(part 1 of 2)
# Autodesk Inventor assembly: Rebuild Shooter Assembly
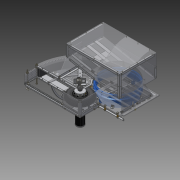
[picture p0: Inventor's stored thumbnail of the model, 180x180]
Saved by Autodesk Inventor 2014 SP1 (Build 180222100, 222)
## iProperties
Created: 2013-10-27
Part Number: Rebuild Shooter Assembly
Document SubType Name: Assembly
Designer: Moses
Mass: 10351.2 g
Surface Area: 36486.6 cm^2
Volume: 5797.69 cm^3
Density: 1.78541 g/cm^3
Author: Moses
## Documents named in this file (107)
- C:\Users\Moses\Documents\Inventor\Rebuilds\Rebuild Sally\Rebuild Shooter Assembly.iam
- C:\Users\Moses\Documents\Inventor\Rebuilds\Rebuild Sally\Spur Gear21.ipt
- C:\Users\Moses\Documents\Inventor\Rebuilds\Rebuild Sally\Bearing Mount 2 v1.ipt
- C:\Users\Moses\Documents\Inventor\Rebuilds\Rebuild Sally\Bearing.ipt
- C:\Users\Moses\Documents\Inventor\Rebuilds\Rebuild Sally\Shorter Shaft.ipt
- C:\Users\Moses\Documents\Inventor\Rebuilds\Rebuild Sally\Rebuild Shooter Main Base.ipt
- C:\Users\Moses\Documents\Inventor\Rebuilds\Rebuild Sally\Gusset 5.ipt
- C:\Users\Moses\Documents\Inventor\Rebuilds\Rebuild Sally\Rebuild L-Channel Strength.ipt
- C:\Users\Moses\Documents\Inventor\Rebuilds\Rebuild Sally\Bearing Mount v1.ipt
- C:\Users\Moses\Documents\Inventor\Rebuilds\Rebuild Sally\Bearing Mount Top.ipt
- C:\Users\Moses\Documents\Inventor\Rebuilds\Rebuild Sally\Rubber Cushion.ipt
- C:\Users\Moses\Documents\Inventor\Rebuilds\Rebuild Sally\CIM Bearing.ipt
- C:\Users\Moses\Documents\Inventor\Rebuilds\Rebuild Sally\Pneumatic Wheel.iam
- C:\Users\Moses\Documents\Inventor\Rebuilds\Rebuild Sally\2469K200.ipt
- C:\Users\Moses\Documents\Inventor\Rebuilds\Rebuild Sally\CIM motor1.ipt
- C:\Users\Moses\Documents\Inventor\Rebuilds\Rebuild Sally\Cim Mount.ipt
- C:\Users\Moses\Documents\Inventor\Rebuilds\Rebuild Sally\Runner Rails v2.ipt
- C:\Users\Moses\Documents\Inventor\Rebuilds\Rebuild Sally\Pneumatic Hub.ipt
- C:\Users\Moses\Documents\Inventor\Rebuilds\Rebuild Sally\0.25x20 Washer.ipt
- C:\Users\Moses\Documents\Inventor\Rebuilds\Rebuild Sally\Standard High-Strength Steel Cap Screw 0.25-20 Thread\Fully Threaded\1.000 in 92620A542\92620A542.ipt
- C:\Users\Moses\Documents\Inventor\Rebuilds\Rebuild Sally\Standard High-Strength Steel Cap Screw 0.25-20 Thread\90630A110.ipt
- C:\Users\Moses\Documents\Inventor\Rebuilds\Rebuild Sally\Standard High-Strength Steel Cap Screw 0.25-20 Thread\Fully Threaded\6.000 in 92620A559\92620A559.ipt
- C:\Users\Moses\Documents\Inventor\Rebuilds\Rebuild Sally\8mm shaft 2.ipt
- C:\Users\Moses\Documents\Inventor\Rebuilds\Rebuild Sally\93330A493.ipt
- C:\Users\Moses\Documents\Inventor\Rebuilds\Rebuild Sally\Standard High-Strength Steel Cap Screw 0.25-20 Thread\Fully Threaded\5.000 in 92620A557\92620A557.ipt
- C:\Users\Moses\Documents\Inventor\Rebuilds\Rebuild Sally\6280K341.ipt
- C:\Users\Moses\Documents\Inventor\Rebuilds\Rebuild Sally\0.5 inch Shaft to 8mm Shaft Insert.ipt
- C:\Users\Moses\Documents\Inventor\Rebuilds\Rebuild Sally\8mm Shaft Spacer 1 Shooter.ipt
- C:\Users\Moses\Documents\Inventor\Rebuilds\Rebuild Sally\Shooter 8mm Key Sprocket Encoder.ipt
- C:\Users\Moses\Documents\Inventor\Rebuilds\Rebuild Sally\Standard High-Strength Steel Cap Screw 0.25-20 Thread\Fully Threaded\4.000 in 92620A555\92620A555.ipt
- C:\Users\Moses\Documents\Inventor\Rebuilds\Rebuild Sally\Shooter Side Support Bar - R.ipt
- C:\Users\Moses\Documents\Inventor\Rebuilds\Rebuild Sally\Shooter Side Support Bar - L.ipt
- C:\Users\Moses\Documents\Inventor\Rebuilds\Rebuild Sally\Shooter Back Support Bar.ipt
- C:\Users\Moses\Documents\Inventor\Rebuilds\Rebuild Sally\Shooter Middle Support Bar.ipt
- C:\Users\Moses\Documents\Inventor\Rebuilds\Rebuild Sally\Drive Base Kit\DBK_0820Spacer_am-2243 (modified).ipt
- C:\Users\Moses\Documents\Inventor\Rebuilds\Rebuild Sally\Drive Base Kit\DBK_0820Spacer_am-2243 (modified 2).ipt
- C:\Users\Moses\Documents\Inventor\Rebuilds\Rebuild Sally\Standard #10 Washer.ipt
- C:\Users\Moses\Documents\Inventor\Rebuilds\Rebuild Sally\10-32 316 Stainless Steel Pan Head Philips Machine Screw\0.500\91735A829.ipt
- C:\Users\Moses\Documents\Inventor\Rebuilds\Rebuild Sally\Wheel Shield 1.ipt
- C:\Users\Moses\Documents\Inventor\Rebuilds\Rebuild Sally\Wheel Shield 2.ipt
- C:\Users\Moses\Documents\Inventor\Rebuilds\Rebuild Sally\Standard High-Strength Steel Cap Screw 0.25-20 Thread\Fully Threaded\1.500 in 92620A546\92620A546.ipt
- C:\Users\Moses\Documents\Inventor\Rebuilds\Rebuild Sally\Standard High-Strength Steel Cap Screw 0.25-20 Thread\Fully Threaded\1.250 in 92620A544\92620A544.ipt
- C:\Users\Moses\Documents\Inventor\Rebuilds\Rebuild Sally\Standard High-Strength Steel Cap Screw 0.25-20 Thread\Fully Threaded\1.750 in 92620A548\92620A548.ipt
- C:\Users\Moses\Documents\Inventor\Rebuilds\Rebuild Sally\0.25x20 Washer Large Diameter.ipt
- C:\Users\Moses\Documents\Inventor\Rebuilds\Rebuild Sally\7547K130.ipt
- C:\Users\Moses\Documents\Inventor\Rebuilds\Rebuild Sally\Hopper Bracing P1.ipt
- C:\Users\Moses\Documents\Inventor\Rebuilds\Rebuild Sally\Shooter I Brace.ipt
- C:\Users\Moses\Documents\Inventor\Rebuilds\Rebuild Sally\Standard High-Strength Steel Cap Screw 0.25-20 Thread\Fully Threaded\0.750 in 92620A540\92620A540.ipt
- C:\Users\Moses\Documents\Inventor\Rebuilds\Rebuild Sally\Standard High-Strength Steel Cap Screw 0.25-20 Thread\Thread Length 0.75 - 1 in\1.250 in 91257A544\91257A544.ipt
- C:\Users\Moses\Documents\Inventor\Rebuilds\Rebuild Sally\Rebuild Outer Rail v1.ipt
- C:\Users\Moses\Documents\Inventor\Rebuilds\Rebuild Sally\Standard High-Strength Steel Cap Screw 0.25-20 Thread\Fully Threaded\0.500 in 92620A537\92620A537.ipt
- C:\Users\Moses\Documents\Inventor\Rebuilds\Rebuild Sally\91831A411.ipt
- C:\Users\Moses\Documents\Inventor\Rebuilds\Rebuild Sally\10-32 316 Stainless Steel Pan Head Philips Machine Screw\0.750\91735A831.ipt
- C:\Users\Moses\Documents\Inventor\Rebuilds\Rebuild Sally\Shooter Magnetic Sensor Mount Bracket.ipt
- C:\Users\Moses\Documents\Inventor\Rebuilds\Rebuild Sally\176_DP_D_229__F_D_231_1__F_D_3556__2_03\7.ipt
- C:\Users\Moses\Documents\Inventor\Rebuilds\Rebuild Sally\Shooter Top Shield.ipt
- C:\Users\Moses\Documents\Inventor\Rebuilds\Rebuild Sally\Shooter Wheel Shields Connector Bar.ipt
- C:\Users\Moses\Documents\Inventor\Rebuilds\Rebuild Sally\Drive Base Kit\DBK_0820Spacer_am-2243 (modified 3).ipt
- C:\Users\Moses\Documents\Inventor\Rebuilds\Rebuild Sally\0.125 Pop Rivet.ipt
- C:\Users\Moses\Documents\Inventor\Rebuilds\Rebuild Sally\Shooter Magnetic Sensor V2.ipt
- C:\Users\Moses\Documents\Inventor\Rebuilds\Rebuild Sally\Hopper Bracing P2.ipt
- C:\Users\Moses\Documents\Inventor\Rebuilds\Rebuild Sally\Hopper Bracing P3.ipt
- C:\Users\Moses\Documents\Inventor\Rebuilds\Rebuild Sally\Hopper Left Side Leg.ipt
- C:\Users\Moses\Documents\Inventor\Rebuilds\Rebuild Sally\Hopper Right Side Leg.ipt
- C:\Users\Moses\Documents\Inventor\Rebuilds\Rebuild Sally\Hopper Bottom.ipt
- C:\Users\Moses\Documents\Inventor\Rebuilds\Rebuild Sally\Hopper Left Side.ipt
- C:\Users\Moses\Documents\Inventor\Rebuilds\Rebuild Sally\Hopper Back Wedge Side.ipt
- C:\Users\Moses\Documents\Inventor\Rebuilds\Rebuild Sally\Hopper Top.ipt
- C:\Users\Moses\Documents\Inventor\Rebuilds\Rebuild Sally\Hopper Bracing Top Left P4.ipt
- C:\Users\Moses\Documents\Inventor\Rebuilds\Rebuild Sally\Hopper Front.ipt
- C:\Users\Moses\Documents\Inventor\Rebuilds\Rebuild Sally\Hopper Right.ipt
- C:\Users\Moses\Documents\Inventor\Rebuilds\Rebuild Sally\Hopper Bracing Front Left P5.ipt
- C:\Users\Moses\Documents\Inventor\Rebuilds\Rebuild Sally\Hopper Bracing Front Bottom P6.ipt
- C:\Users\Moses\Documents\Inventor\Rebuilds\Rebuild Sally\Hopper Bracing Front Right P7.ipt
- C:\Users\Moses\Documents\Inventor\Rebuilds\Rebuild Sally\Hopper Bracing Front Top P8.ipt
- C:\Users\Moses\Documents\Inventor\Rebuilds\Rebuild Sally\Hopper Bracing Right Bottom P9.ipt
- C:\Users\Moses\Documents\Inventor\Rebuilds\Rebuild Sally\Hopper Bracing Right Top P10.ipt
- C:\Users\Moses\Documents\Inventor\Rebuilds\Rebuild Sally\Hopper Teflon Strip P1.ipt
- C:\Users\Moses\Documents\Inventor\Rebuilds\Rebuild Sally\Hopper Teflon Strip P2.ipt
- C:\Users\Moses\Documents\Inventor\Rebuilds\Rebuild Sally\Hopper Teflon Strip P3.ipt
- C:\Users\Moses\Documents\Inventor\Rebuilds\Rebuild Sally\Hopper Teflon Strip P4.ipt
- C:\Users\Moses\Documents\Inventor\Rebuilds\Rebuild Sally\Hopper Bracing Back Bottom P11.ipt
- C:\Users\Moses\Documents\Inventor\Rebuilds\Rebuild Sally\Hopper Bracing Back Left P12.ipt
- C:\Users\Moses\Documents\Inventor\Rebuilds\Rebuild Sally\Hopper Bracing Right Leg P13.ipt
- C:\Users\Moses\Documents\Inventor\Rebuilds\Rebuild Sally\Hopper Bouncer Mounting Brace P1.ipt
- C:\Users\Moses\Documents\Inventor\Rebuilds\Rebuild Sally\Bounce Polycarbonate Flap.ipt
- C:\Users\Moses\Documents\Inventor\Rebuilds\Rebuild Sally\Hopper Bracing P12 to P1.ipt
- C:\Users\Moses\Documents\Inventor\Rebuilds\Rebuild Sally\Hopper Pail Mounting Brace P13.ipt
- C:\Users\Moses\Documents\Inventor\Rebuilds\Rebuild Sally\Trimmed Leaktite 3.5-Gal. Blue Plastic Translucent Pail Hopper V3.ipt
- C:\Users\Moses\Documents\Inventor\Rebuilds\Rebuild Sally\Hopper Teflon Strip P5.ipt
- C:\Users\Moses\Documents\Inventor\Rebuilds\Rebuild Sally\Hopper Teflon Strip P6.ipt
- C:\Users\Moses\Documents\Inventor\Rebuilds\Rebuild Sally\Hopper to Pail Polycarbonate Flap Connector V2.ipt
- C:\Users\Moses\Documents\Inventor\Rebuilds\Rebuild Sally\90715A007.ipt
- C:\Users\Moses\Documents\Inventor\Rebuilds\Rebuild Sally\Drive Base Kit\DBK_0820Spacer_am-2243 (modified for Shooter Shaft Spacer 1).ipt
- C:\Users\Moses\Documents\Inventor\Rebuilds\Rebuild Sally\Drive Base Kit\DBK_0820Spacer_am-2243 (modified for Shooter Shaft Spacer 2).ipt
- C:\Users\Moses\Documents\Inventor\Rebuilds\Rebuild Sally\10-32 Black-Oxide Alloy Steel Socket Head Cap Screw\0.7500\91251A345.ipt
- C:\Users\Moses\Documents\Inventor\Rebuilds\Rebuild Sally\10-32 Black-Oxide Alloy Steel Socket Head Cap Screw\2.5000\91251A355.ipt
- C:\Users\Moses\Documents\Inventor\Rebuilds\Rebuild Sally\Shooter 8mm Key Primary Wheel.ipt
- C:\Users\Moses\Documents\Inventor\Rebuilds\Rebuild Sally\Rebuild Shooter NCDME075-0600 Cylinder Mounting Bracket.ipt
- C:\Users\Moses\Documents\Inventor\Rebuilds\Rebuild Sally\NCDME075-0600 SMC Pneumatic Cylinder.iam
- C:\Users\Moses\Documents\Inventor\Rebuilds\Rebuild Sally\94846A535.ipt
- C:\Users\Moses\Documents\Inventor\Rebuilds\Rebuild Sally\Rebuild Puller Hook.ipt
- C:\Users\Moses\Documents\Inventor\Rebuilds\Rebuild Sally\Standard #4 Washer.ipt
- C:\Users\Moses\Documents\Inventor\Rebuilds\Rebuild Sally\4-40 18-8 Stainless Steel Pan Head Phillips Machine Screw\18-8 Stainless Steel Nylon-Insert Hex Locknut\91831A005.ipt
- C:\Users\Moses\Documents\Inventor\Rebuilds\Rebuild Sally\4-40 18-8 Stainless Steel Pan Head Phillips Machine Screw\0.6250\91772A112.ipt
- C:\Users\Moses\Documents\Inventor\Rebuilds\Rebuild Sally\4-40 18-8 Stainless Steel Pan Head Phillips Machine Screw\0.5000\91772A110.ipt
- C:\Users\Moses\Documents\Inventor\Rebuilds\Rebuild Sally\4-40 18-8 Stainless Steel Pan Head Phillips Machine Screw\0.7500\91772A113.ipt
## Components (473 placed, 106 different names)
1. Shooter Wheel Shields Connector Bar:1 — Mate:124, Mate:125, Flush:76, Mate:89, Mate:128
2. Shooter Top Shield:1 — Flush:73, Mate:123, Flush:74, Flush:75, Insert:58, Insert:57, Mate:119, Mate:188, Flush:163
3. Shooter Magnetic Sensor Mount Bracket:1 — Mate:119, Angle:74, Mate:120, Mate:121, Insert:177, Insert:178
4. DBK_0820Spacer_am-2243 (modified 3):1 — Insert:196
5. 93330A493:1 — Insert:75
6. 7547K130:3 — Mate:101, Mate:102, Mate:103
7. 7547K130:1 — Mate:98, Mate:99, Mate:100
8. Shooter I Brace:1 — Mate:105, Flush:18, Mate:109, Mate:111, Mate:113, Flush:175, Insert:390, Insert:392, Insert:393, Insert:394
9. Shooter Side Support Bar - R:1 — Mate:84, Tangent:86, Flush:6, Mate:86, Flush:8, Insert:78, Insert:114, Insert:115, Insert:135
10. Shooter Side Support Bar - L:1 — Mate:85, Flush:7, Tangent:87, Insert:92, Insert:100, Mate:128, Insert:305, Insert:361, Mate:228, Mate:229, Flush:176
11. Shooter Middle Support Bar:1 — Flush:14, Mate:93, Insert:85, Insert:87, Mate:57, Insert:45, Insert:103, Insert:104, Insert:164
12. Shooter Back Support Bar:1 — Mate:86, Tangent:88, Flush:8, Mate:40, Insert:130, Flush:151, Flush:174
13. Wheel Shield 2:1 — Mate:89, Flush:10, Mate:90, Flush:11, Mate:124, Flush:76, Insert:201, Insert:202
14. Wheel Shield 1:1 — Mate:88, Flush:9, Flush:10, Mate:90, Flush:11, Mate:125, Insert:199, Insert:200
15. Rubber Cushion:1 — Mate:48, Mate:49, Flush:3
16. Bearing:2 — Mate:19, Mate:103
17. Bearing:1 — Mate:100
18. Spur Gear2:1 — Mate:20, Mate:21, Mate:22, Mate:23, Mate:24, Mate:25, Mate:27, Mate:28, Mate:29, Mate:30, Mate:31, Mate:32, Insert:395, Insert:396
19. Shorter Shaft:1 — Mate:19, Mate:98, Mate:99, Mate:101, Mate:102
20. Runner Rails v2:1 — Mate:59, Mate:60, Mate:61, Insert:84, Flush:14, Insert:86, Insert:88, Insert:101, Insert:102, Mate:104, Mate:220, Flush:17, Insert:171, Insert:172, Insert:173, Insert:174, Insert:175, Insert:176, Mate:130, Mate:132, Flush:78, Mate:133, Mate:135, Mate:152, Mate:200, Tangent:94, Flush:165, Mate:202, Mate:205, Mate:206, Mate:221
21. Cim Mount:1 — Insert:9, Mate:55, Mate:56, Mate:57, Mate:58, Insert:22, Insert:23, Insert:34, Insert:35, Insert:40, Insert:71, Insert:72, Insert:75, Mate:93, Insert:93, Insert:116, Insert:117, Insert:163, Insert:363, Insert:364
22. Bearing Mount Top:1 — Mate:45, Mate:46, Mate:47, Insert:7, Mate:50, Insert:56, Angle:74, Mate:120, Mate:121, Mate:122, Flush:73, Mate:123, Flush:74, Flush:75, Mate:153
23. Rebuild Outer Rail v1:1 — Mate:42, Mate:44, Mate:45, Mate:46, Mate:48, Insert:51, Insert:53, Insert:55, Insert:69, Mate:114, Flush:65, Flush:66
24. Rebuild Outer Rail v1:2 — Mate:114, Flush:65, Flush:66, Mate:115, Flush:67, Flush:70
25. Rebuild Outer Rail v1:3 — Mate:115, Mate:116, Flush:67, Flush:68, Flush:70, Flush:71
26. Rebuild Outer Rail v1:4 — Mate:116, Mate:117, Flush:68, Flush:69, Flush:71, Flush:72
27. Rebuild Outer Rail v1:5 — Mate:117, Flush:69, Flush:72, Mate:118, Mate:222
28. Bearing Mount v1:1 — Mate:39, Mate:40, Flush:2, Mate:41, Mate:44, Mate:49, Flush:3, Insert:8, Mate:59, Mate:60, Mate:61, Insert:66, Insert:94, Mate:118, Insert:165, Insert:166, Insert:167, Insert:168, Insert:169, Insert:170
29. Rebuild L-Channel Strength:1 — Mate:36, Mate:37, Mate:38, Mate:88, Flush:9, Insert:121, Insert:125, Mate:127, Insert:208, Insert:303, Insert:304
30. Gusset 5:4 — Mate:27, Mate:31, Mate:32, Insert:146, Insert:153
31. Gusset 5:3 — Mate:28, Mate:29, Mate:30, Mate:33, Insert:141, Insert:152
32. Gusset 5:2 — Mate:23, Mate:24, Mate:25, Mate:34, Mate:35, Insert:145, Insert:150
33. Gusset 5:1 — Mate:20, Mate:21, Mate:22, Insert:147, Insert:151
34. Bearing Mount 2 v1:1 — Mate:8, Mate:9, Mate:10, Mate:14, Insert:139
35. Bearing Mount 2 v1:2 — Mate:11, Mate:12, Mate:13, Insert:133, Insert:137
36. Rebuild Shooter Main Base:1 — Mate:11, Mate:12, Mate:8, Mate:9, Mate:10, Mate:13, Mate:14, Mate:33, Mate:34, Mate:35, Mate:36, Mate:37, Mate:38, Mate:39, Flush:2, Mate:41, Mate:42, Mate:55, Mate:56, Insert:65, Mate:74, Insert:76, Mate:84, Flush:6, Mate:85, Flush:7, Insert:44, Insert:112, Insert:122, Mate:105, Flush:18, Insert:148, Insert:149, Mate:106, Mate:107, Mate:108, Mate:110, Mate:112, Mate:126, Insert:196, Insert:207, Insert:39, Angle:79, Angle:80
37. Shooter 8mm Key Primary Wheel:1 — Flush:173, Mate:225, Mate:226, Mate:227
38. DBK_0820Spacer_am-2243 (modified for Shooter Shaft Spacer 1):1 — Insert:358
39. DBK_0820Spacer_am-2243 (modified for Shooter Shaft Spacer 2):1 — Insert:359
40. Shooter Magnetic Sensor V2:1 — Insert:177
41. 6280K341:1 — Mate:77, Flush:5, Angle:3, Mate:78
42. 0.5 inch Shaft to 8mm Shaft Insert:1 — Mate:75, Mate:76, Mate:77, Flush:5, Angle:3
43. 8mm Shaft Spacer 1 Shooter:1 — Mate:79, Mate:80, Mate:78, Mate:83
44. Shooter 8mm Key Sprocket Encoder:1 — Mate:81, Mate:82, Mate:83
45. 8mm shaft 2:1 — Mate:51, Mate:52, Mate:54, Rotation:1, Mate:66, Mate:67, Mate:68, Mate:69, Mate:75, Mate:76, Mate:79, Mate:81, Mate:82, Mate:226
46. Pneumatic Wheel:1 [sub-assembly] — Mate:50, Mate:70, Mate:71, Mate:72
47. 2469K200:1 — Mate:52, Mate:53, Flush:4, Rotation:1
48. CIM motor1:1 — Mate:53, Mate:54, Flush:4, Insert:9, Mate:58
49. Pneumatic Hub:1 — Mate:66, Mate:69, Mate:71, Insert:368, Insert:374, Insert:375, Insert:376, Insert:377, Insert:378
50. Pneumatic Hub:2 — Mate:67, Mate:68, Mate:70, Mate:72, Insert:188, Insert:189, Insert:190, Insert:191, Insert:192, Insert:193, Mate:122, Insert:359, Flush:173, Mate:225, Mate:227
51. CIM Bearing:2 — Insert:8, Insert:358
52. CIM Bearing:1 — Insert:7, Mate:51, Mate:80
53. 90630A110:37 — Insert:391
54. 0.25x20 Washer:100 — Insert:127, Insert:392
55. 0.25x20 Washer:102 — Insert:129, Insert:394
56. 0.25x20 Washer:101 — Insert:128, Insert:393
57. Standard #4 Washer:1 — Insert:395, Insert:398
58. Standard #4 Washer:2 — Insert:396, Insert:397
59. 91772A112:1 — Insert:398
60. 91831A005:1 — Insert:397
61. 90630A110:36
62. 0.25x20 Washer:98 — Insert:388
63. 91257A544:5 — Insert:389
64. 0.25x20 Washer:99 — Insert:389, Insert:390
65. 94846A535:1 — Insert:386
66. 91831A005:8 — Insert:379
67. Standard #4 Washer:14 — Insert:379
68. 91831A005:7 — Insert:380
69. Standard #4 Washer:13 — Insert:380
70. 91772A113:2
71. 91772A113:1
72. Standard #10 Washer:12 — Insert:364, Insert:365
73. Standard #10 Washer:13 — Insert:363, Insert:366
74. 91251A345:1 — Insert:366
75. 91251A345:2 — Insert:365
76. 91251A355:1 — Insert:367
77. Standard #10 Washer:14 — Insert:367, Insert:368
78. 91251A355:2
79. Standard #10 Washer:15 — Insert:374
80. 91251A355:3
81. Standard #10 Washer:16 — Insert:375
82. 91251A355:4
83. Standard #10 Washer:17 — Insert:376
84. 91251A355:5
85. 91251A355:6
86. Standard #10 Washer:18 — Insert:378
87. Standard #10 Washer:19 — Insert:377
88. DBK_0820Spacer_am-2243 (modified):1 — Insert:89, Mate:92
89. DBK_0820Spacer_am-2243 (modified 2):1 — Insert:91
90. DBK_0820Spacer_am-2243 (modified):2 — Insert:90
91. DBK_0820Spacer_am-2243 (modified 2):2 — Insert:362
92. 91257A544:4
93. 0.25x20 Washer:97 — Insert:361
94. 0.125 Pop Rivet:91 — Mate:224, Tangent:211
95. 91831A005:13 — Insert:303
96. 91831A005:14 — Insert:304
97. 91772A110:8
98. 90715A007:3 — Insert:305
99. 91772A110:9
100. 91772A110:10
101. 91831A005:15 — Insert:309
102. Standard #4 Washer:33 — Insert:309
103. 91831A005:16 — Insert:310
104. Standard #4 Washer:34 — Insert:310
105. 91831A005:17 — Insert:313
106. Standard #4 Washer:35 — Insert:313
107. 91831A005:18 — Insert:314
108. Standard #4 Washer:36 — Insert:314
109. 91831A005:19 — Insert:315
110. Standard #4 Washer:37 — Insert:315
111. 91772A112:4
112. 91772A112:5
113. 91772A112:6
114. 91772A112:7
115. 91772A112:8
116. 91831A005:9 — Insert:324
117. Standard #4 Washer:20 — Insert:324, Insert:328
118. 91831A005:10 — Insert:325
119. Standard #4 Washer:21 — Insert:325, Insert:329
120. 91831A005:11 — Insert:326
121. Standard #4 Washer:22 — Insert:326, Insert:330
122. 91831A005:12 — Insert:327
123. Standard #4 Washer:23 — Insert:327, Insert:331
124. 91772A110:7
125. 91772A110:6
126. 91772A110:5
127. 91772A110:4
128. 91257A544:3 — Insert:336
129. 91831A005:4 — Insert:337
130. Standard #4 Washer:5 — Insert:337, Insert:340
131. 91831A005:5 — Insert:338
132. Standard #4 Washer:4 — Insert:338, Insert:341
133. 91831A005:6 — Insert:339
134. Standard #4 Washer:3 — Insert:339, Insert:342
135. 91772A110:1
136. 91772A110:2
137. 91772A110:3
138. 91831A005:2 — Insert:346
139. Standard #4 Washer:11 — Insert:346
140. 91831A005:3 — Insert:348
141. Standard #4 Washer:12 — Insert:348
142. 91772A112:2
143. 91831A005:21
144. 91772A112:3
145. Standard #4 Washer:39
146. 91831A005:20
147. Standard #4 Washer:38
148. 91772A112:10
149. 91772A112:9
150. 0.125 Pop Rivet:90 — Mate:217, Tangent:209
151. 0.125 Pop Rivet:87 — Insert:302, Mate:218
152. 0.125 Pop Rivet:88 — Insert:301, Mate:219
153. 0.125 Pop Rivet:89 — Mate:216, Tangent:208
154. 0.125 Pop Rivet:85 — Insert:299, Mate:205
155. 0.125 Pop Rivet:86 — Insert:300
156. 0.125 Pop Rivet:78 — Insert:292, Mate:197
157. 0.125 Pop Rivet:79 — Insert:293
158. 0.125 Pop Rivet:81 — Insert:295
159. 0.125 Pop Rivet:80 — Insert:294, Mate:198
160. 0.125 Pop Rivet:82 — Insert:296
161. 0.125 Pop Rivet:84 — Insert:297
162. 0.125 Pop Rivet:83 — Insert:298
163. Standard #4 Washer:6 — Insert:277
164. Standard #4 Washer:7 — Insert:278
165. Standard #4 Washer:8 — Insert:279
166. Standard #4 Washer:10
167. Standard #4 Washer:9
168. Standard #4 Washer:30
169. Standard #4 Washer:32
170. Standard #4 Washer:31 — Insert:284
171. Standard #4 Washer:29 — Insert:286
172. Standard #4 Washer:25
173. Standard #4 Washer:26
174. Standard #4 Washer:27
175. Standard #4 Washer:28 — Insert:291
176. Standard #4 Washer:24 — Insert:290
177. 0.125 Pop Rivet:76 — Insert:275
178. 0.125 Pop Rivet:77 — Insert:276
179. 0.125 Pop Rivet:68 — Insert:267
180. 0.125 Pop Rivet:69 — Insert:268
181. 0.125 Pop Rivet:70 — Insert:269
182. 0.125 Pop Rivet:71 — Insert:270
183. 0.125 Pop Rivet:72 — Insert:271
184. 0.125 Pop Rivet:73 — Insert:272
185. 0.125 Pop Rivet:75 — Insert:274
186. 0.125 Pop Rivet:74 — Insert:273
187. 0.125 Pop Rivet:47 — Mate:179, Tangent:92
188. 0.125 Pop Rivet:46 — Mate:178, Tangent:93
189. 0.125 Pop Rivet:48 — Mate:180, Tangent:91
190. 0.125 Pop Rivet:49 — Mate:181, Tangent:90
191. 0.125 Pop Rivet:50 — Mate:182, Tangent:89
192. 0.125 Pop Rivet:52 — Insert:251
193. 0.125 Pop Rivet:51 — Insert:250
194. 0.125 Pop Rivet:53 — Insert:252
195. 0.125 Pop Rivet:54 — Insert:253
196. 0.125 Pop Rivet:55 — Insert:254
197. 0.125 Pop Rivet:57 — Insert:256
198. 0.125 Pop Rivet:56 — Insert:255
199. 0.125 Pop Rivet:59 — Insert:258
200. 0.125 Pop Rivet:58 — Insert:257
201. 0.125 Pop Rivet:61 — Insert:260
202. 0.125 Pop Rivet:60 — Insert:259
203. 0.125 Pop Rivet:63 — Insert:262
204. 0.125 Pop Rivet:62 — Insert:261
205. 0.125 Pop Rivet:64 — Insert:263
206. 0.125 Pop Rivet:65 — Insert:264
207. 0.125 Pop Rivet:67 — Insert:266
208. 0.125 Pop Rivet:66 — Insert:265
209. 0.125 Pop Rivet:23 — Insert:227
210. 0.125 Pop Rivet:24 — Insert:228
211. 0.125 Pop Rivet:25 — Insert:229
212. 0.125 Pop Rivet:26 — Insert:230
213. 0.125 Pop Rivet:27 — Insert:231
214. 0.125 Pop Rivet:29 — Insert:233
215. 0.125 Pop Rivet:28 — Insert:232
216. 0.125 Pop Rivet:30 — Insert:234
217. 0.125 Pop Rivet:31 — Insert:235
218. 0.125 Pop Rivet:32 — Insert:236
219. 0.125 Pop Rivet:34 — Insert:238
220. 0.125 Pop Rivet:33 — Insert:237
221. 0.125 Pop Rivet:35 — Insert:239
222. 0.125 Pop Rivet:36 — Insert:240
223. 0.125 Pop Rivet:37 — Insert:241
224. 0.125 Pop Rivet:38 — Insert:242
225. 0.125 Pop Rivet:39 — Insert:243
226. 0.125 Pop Rivet:40 — Insert:244
227. 0.125 Pop Rivet:41 — Insert:245
228. 0.125 Pop Rivet:42 — Insert:246
229. 0.125 Pop Rivet:43 — Insert:247
230. 0.125 Pop Rivet:44 — Insert:248
231. 0.125 Pop Rivet:45 — Insert:249
232. 0.125 Pop Rivet:19 — Insert:223
233. 0.125 Pop Rivet:20 — Insert:224
234. 0.125 Pop Rivet:21 — Insert:225
235. 0.125 Pop Rivet:22 — Insert:226
236. 0.125 Pop Rivet:11 — Insert:215
237. 0.125 Pop Rivet:12 — Insert:216
238. 0.125 Pop Rivet:13 — Insert:217
239. 0.125 Pop Rivet:15 — Insert:219
240. 0.125 Pop Rivet:14 — Insert:218
241. 0.125 Pop Rivet:16 — Insert:220
242. 0.125 Pop Rivet:17 — Insert:221
243. 0.125 Pop Rivet:18 — Insert:222
244. 0.125 Pop Rivet:6 — Insert:210
245. 0.125 Pop Rivet:7 — Insert:211
246. 0.125 Pop Rivet:8 — Insert:212
247. 0.125 Pop Rivet:9 — Insert:213
248. 0.125 Pop Rivet:10 — Insert:214
249. 90630A110:35 — Insert:208
250. 0.25x20 Washer:96 — Insert:207, Insert:209
251. 92620A540:11 — Insert:209
252. Standard #4 Washer:40
253. Standard #4 Washer:41
254. 0.25x20 Washer:95 — Mate:126, Mate:127, Insert:194
255. 90630A110:34 — Insert:194
256. 92620A540:10 — Insert:195
257. Standard #4 Washer:18
258. Standard #4 Washer:19
259. 0.125 Pop Rivet:1 — Insert:199
260. 0.125 Pop Rivet:2 — Insert:200
261. 0.125 Pop Rivet:3 — Insert:201
262. 0.125 Pop Rivet:4 — Insert:202
263. 0.125 Pop Rivet:5 — Insert:204, Tangent:207
264. Standard #4 Washer:17
265. Standard #10 Washer:6 — Insert:182, Insert:188
266. Standard #10 Washer:7 — Insert:183, Insert:189
267. Standard #10 Washer:8 — Insert:184, Insert:190
268. Standard #10 Washer:9 — Insert:185, Insert:191
269. Standard #10 Washer:10 — Insert:186, Insert:192
270. Standard #10 Washer:11 — Insert:187, Insert:193
271. 91831A411:7 — Insert:182
272. 91831A411:8 — Insert:183
273. 91831A411:9 — Insert:184
274. 91831A411:10 — Insert:185
275. 91831A411:11 — Insert:186
276. 91831A411:12 — Insert:187
277. Standard #4 Washer:15
278. Standard #4 Washer:16
279. 7:1 — Insert:178, Insert:179
280. 7:2 — Insert:179
281. 91735A831:1 — Insert:171
282. 91735A831:2 — Insert:172
283. 91735A831:3 — Insert:173
284. 91735A831:4 — Insert:174
285. 91735A831:5 — Insert:176
286. 91735A831:6 — Insert:175
287. 90630A110:33 — Insert:163
288. 92620A537:1 — Insert:164
289. 91831A411:1 — Insert:165
290. 91831A411:2 — Insert:166
291. 91831A411:3 — Insert:167
292. 91831A411:4 — Insert:168
293. 91831A411:5 — Insert:169
294. 91831A411:6 — Insert:170
295. 91257A544:2 — Insert:162
296. 91257A544:1 — Insert:161
297. 92620A540:9
298. 0.25x20 Washer:94 — Mate:112, Mate:113
299. 92620A540:8
300. 0.25x20 Washer:93 — Mate:110, Mate:111
301. 92620A540:7
302. 0.25x20 Washer:92 — Mate:108, Mate:109
303. 92620A555:1 — Insert:77
304. 90630A110:27
305. 90630A110:28
306. 90630A110:29
307. 90630A110:30
308. 90630A110:31
309. 90630A110:32
310. 92620A540:3 — Insert:154
311. 92620A540:4 — Insert:155
312. 92620A540:5 — Insert:156
313. 92620A540:6 — Insert:157
314. 90630A110:13 — Insert:105
315. 90630A110:14 — Insert:106
316. 92620A546:1 — Insert:107
317. 92620A546:2 — Insert:108
318. 92620A544:1 — Insert:109
319. 90630A110:15 — Insert:113
320. 90630A110:16 — Insert:118
321. 90630A110:17 — Insert:119
322. 90630A110:19 — Insert:121
323. 90630A110:23 — Insert:127
324. 90630A110:24 — Insert:128
325. 90630A110:25 — Insert:129
326. 90630A110:26 — Insert:131
327. 92620A540:1 — Insert:132
328. 92620A540:2
329. 0.25x20 Washer:68 — Insert:110
330. 0.25x20 Washer:69 — Insert:111
331. 0.25x20 Washer:70 — Insert:112, Insert:113
332. 0.25x20 Washer:71 — Insert:114, Insert:161
333. 0.25x20 Washer:72 — Insert:115, Insert:162
334. 0.25x20 Washer:74 — Insert:117, Insert:119
335. 0.25x20 Washer:73 — Insert:116, Insert:118
336. 92620A548:1 — Insert:122
337. 0.25x20 Washer Large Diameter:1 — Insert:123, Insert:124, Insert:125
338. 90630A110:20 — Insert:123
339. 90630A110:21 — Insert:124
340. 0.25x20 Washer:75 — Insert:130, Insert:132
341. 0.25x20 Washer:76 — Insert:133, Insert:131
342. 0.25x20 Washer:77 — Insert:135
343. 0.25x20 Washer:78 — Insert:137
344. 0.25x20 Washer:79 — Insert:139
345. 0.25x20 Washer:80 — Insert:141
346. 0.25x20 Washer:81 — Insert:145
347. 0.25x20 Washer:82 — Insert:146
348. 0.25x20 Washer:83 — Insert:147
349. 0.25x20 Washer:84 — Insert:148, Insert:157
350. 0.25x20 Washer:85 — Insert:149, Insert:156
351. 0.25x20 Washer:86 — Mate:107, Insert:155
352. 0.25x20 Washer:87 — Mate:106, Insert:154
353. 0.25x20 Washer:88 — Insert:151, Insert:49
354. 0.25x20 Washer:89 — Insert:150, Insert:48
355. 0.25x20 Washer:90 — Insert:152, Insert:47
356. 0.25x20 Washer:91 — Insert:153, Insert:46
357. Standard #10 Washer:1 — Insert:93, Insert:95
358. Standard #10 Washer:2 — Insert:94, Insert:96
359. 0.25x20 Washer:62 — Insert:92, Insert:336
360. 0.25x20 Washer:64 — Insert:101, Insert:107
361. 0.25x20 Washer:63 — Insert:100, Insert:195
362. 0.25x20 Washer:65 — Insert:102, Insert:108
363. 0.25x20 Washer:67 — Insert:104, Insert:106
364. 0.25x20 Washer:66 — Insert:103, Insert:105
365. 0.25x20 Washer:57 — Insert:84, Insert:109
366. 91735A829:1 — Insert:95
367. 91735A829:2 — Insert:96
368. 0.25x20 Washer:58 — Insert:85, Insert:89
369. 0.25x20 Washer:59 — Insert:86, Mate:92
370. 0.25x20 Washer:60 — Insert:87, Insert:90
371. 0.25x20 Washer:61 — Insert:88
372. 0.25x20 Washer:52 — Insert:78, Insert:79
373. 0.25x20 Washer:53 — Insert:79, Insert:80
374. 0.25x20 Washer:54 — Insert:80, Insert:81
375. 0.25x20 Washer:55 — Insert:81, Insert:82
376. 0.25x20 Washer:56 — Insert:82
377. 90630A110:10 — Insert:73
378. 90630A110:9 — Insert:70
379. 90630A110:11 — Insert:74
380. 0.25x20 Washer:49 — Insert:72, Insert:74
381. 0.25x20 Washer:50 — Insert:71, Insert:73
382. 0.25x20 Washer:51 — Insert:76, Insert:77
383. 92620A559:1 — Insert:65
384. 92620A557:1
385. 0.25x20 Washer:47 — Insert:66
386. 92620A557:2
387. 0.25x20 Washer:46 — Mate:73, Mate:74, Tangent:88
388. 0.25x20 Washer:48 — Insert:69, Insert:70
389. 90630A110:8 — Insert:63
390. 90630A110:7 — Insert:64
391. 90630A110:6 — Insert:61
392. 90630A110:4 — Insert:59
393. 90630A110:3 — Insert:60, Mate:47
394. 90630A110:5 — Insert:62
395. 0.25x20 Washer:45 — Insert:58, Insert:59
396. 0.25x20 Washer:43 — Insert:56, Insert:64
397. 0.25x20 Washer:44 — Insert:57, Insert:62
398. 0.25x20 Washer:42 — Insert:60
399. 0.25x20 Washer:41 — Insert:55
400. 0.25x20 Washer:40 — Insert:61
401. 0.25x20 Washer:39 — Insert:53
402. 0.25x20 Washer:38 — Insert:50, Insert:63
403. 0.25x20 Washer:37 — Insert:50, Insert:51, Mate:73
404. 90630A110:2 — Insert:48
405. 90630A110:1 — Insert:49
406. 92620A542:2 — Insert:47
407. 92620A542:1 — Insert:46
408. 0.25x20 Washer:17 — Insert:30, Insert:110
409. 0.25x20 Washer:18 — Insert:26, Insert:111
410. 0.25x20 Washer:19 — Insert:26, Insert:27
411. 0.25x20 Washer:20 — Insert:27, Insert:28
412. 0.25x20 Washer:21 — Insert:28, Insert:29
413. 0.25x20 Washer:22 — Insert:29, Insert:35
414. 0.25x20 Washer:23 — Insert:30, Insert:31, Tangent:86
415. 0.25x20 Washer:24 — Insert:31, Insert:32
416. 0.25x20 Washer:25 — Insert:32, Insert:33
417. 0.25x20 Washer:26 — Insert:33, Insert:34
418. 0.25x20 Washer:27 — Insert:40, Insert:362
419. 0.25x20 Washer:31 — Insert:39, Tangent:87
420. 0.25x20 Washer:32 — Insert:45, Insert:91
421. 0.25x20 Washer:36 — Insert:44
422. 0.25x20 Washer:1 — Insert:14, Insert:15
423. 0.25x20 Washer:2 — Insert:15, Insert:16
424. 0.25x20 Washer:3 — Insert:14
425. 0.25x20 Washer:4 — Insert:13, Insert:19
426. 0.25x20 Washer:5 — Insert:12, Insert:13
427. 0.25x20 Washer:6 — Insert:10
428. 0.25x20 Washer:7 — Insert:10, Insert:11
429. 0.25x20 Washer:8 — Insert:11, Insert:12
430. 0.25x20 Washer:9 — Insert:17, Insert:18
431. 0.25x20 Washer:10 — Insert:16, Insert:17
432. 0.25x20 Washer:11 — Insert:19, Insert:21
433. 0.25x20 Washer:12 — Insert:18, Insert:20
434. 0.25x20 Washer:14 — Insert:20, Insert:22
435. 0.25x20 Washer:13 — Insert:21, Insert:23
436. Rebuild Puller Hook:1 — Mate:230, Flush:177, Angle:80, Insert:391
437. NCDME075-0600 SMC Pneumatic Cylinder:1 [sub-assembly] — Insert:385, Angle:79, Flush:175, Insert:388, Flush:176, Mate:230, Flush:177
438. Rebuild Shooter NCDME075-0600 Cylinder Mounting Bracket:1 — Mate:228, Mate:229, Insert:385, Flush:174, Insert:386
439. Hopper to Pail Polycarbonate Flap Connector V2:1 — Mate:213, Insert:301, Insert:302, Angle:76, Mate:214, Angle:77, Mate:215, Angle:78
440. Hopper Pail Mounting Brace P13:1 — Mate:202, Tangent:203, Mate:203, Mate:204, Insert:299, Angle:75, Flush:168
441. Hopper Pail Mounting Brace P13:2 — Mate:206, Tangent:204, Mate:207, Angle:75, Insert:300, Flush:167
442. Hopper Teflon Strip P5:1 — Mate:208, Mate:209, Flush:166
443. Hopper Teflon Strip P6:1 — Mate:210, Mate:211, Flush:166, Mate:212
444. Hopper Bracing P12 to P1:1 — Tangent:202, Mate:201, Tangent:207, Mate:223, Flush:170, Flush:171, Flush:172
445. Trimmed Leaktite 3.5-Gal. Blue Plastic Translucent Pail Hopper V3:1 — Mate:200, Tangent:94, Flush:165, Tangent:202, Tangent:203, Mate:204, Tangent:204, Mate:207, Mate:214, Flush:167, Mate:216, Tangent:208, Flush:168, Mate:217, Tangent:209, Mate:218, Flush:172, Mate:224, Tangent:211
446. Hopper Bouncer Mounting Brace P1:1 — Mate:191, Mate:194, Flush:164, Insert:296, Insert:297
447. Hopper Bouncer Mounting Brace P1:2 — Mate:190, Mate:194, Mate:195, Mate:196, Flush:164, Insert:295, Insert:298
448. Bounce Polycarbonate Flap:1 — Insert:292, Insert:293, Insert:294, Mate:199
449. Hopper Bracing Back Bottom P11:1 — Mate:183, Mate:184, Mate:187
450. Hopper Bracing Back Left P12:1 — Mate:185, Mate:186, Flush:162, Mate:187
451. Hopper Bracing Right Leg P13:1 — Mate:188, Mate:189, Flush:163, Mate:138, Insert:340, Insert:341, Insert:342
452. Hopper Teflon Strip P1:1 — Mate:170, Flush:157, Mate:171
453. Hopper Teflon Strip P2:1 — Mate:172, Flush:158, Mate:173
454. Hopper Teflon Strip P3:1 — Mate:174, Flush:159, Mate:175, Mate:211, Mate:212
455. Hopper Teflon Strip P4:1 — Mate:176, Flush:160, Mate:177, Mate:209
456. Hopper Front:1 — Mate:147, Mate:156, Mate:148, Mate:150, Flush:87, Mate:155, Mate:158, Mate:160, Mate:164, Insert:252, Insert:253, Insert:254, Insert:255, Insert:256, Insert:257, Insert:258, Insert:259, Insert:260, Insert:261, Insert:262, Insert:263, Mate:190, Mate:191, Mate:213, Mate:219
457. Hopper Right:1 — Mate:167, Flush:87, Mate:161, Flush:154, Mate:165, Mate:168, Mate:150, Mate:151, Insert:227, Insert:228, Insert:229, Insert:230, Insert:231, Insert:232, Insert:233, Insert:234, Insert:235, Insert:236, Insert:237, Insert:238, Insert:239, Insert:240, Insert:241, Insert:242, Insert:250, Insert:251, Mate:195, Angle:77
458. Hopper Bracing Front Left P5:1 — Mate:154, Mate:155, Flush:152
459. Hopper Bracing Front Right P7:1 — Mate:160, Mate:161, Mate:162
460. Hopper Bracing Front Bottom P6:1 — Mate:158, Mate:159, Flush:153
461. Hopper Bracing Front Top P8:1 — Mate:163, Mate:164, Flush:154, Mate:148
462. Hopper Bracing Right Bottom P9:1 — Mate:165, Mate:166, Flush:155, Flush:161
463. Hopper Bracing Right Top P10:1 — Mate:168, Mate:169, Flush:156
464. Hopper Bracing Top Left P4:1 — Mate:145, Mate:146, Mate:144, Mate:157
465. Hopper Right Side Leg:1 — Mate:138, Mate:153, Mate:151, Flush:155, Flush:156, Mate:189, Insert:277, Insert:278, Insert:279
466. Hopper Bottom:1 — Flush:81, Mate:141, Flush:82, Mate:143, Mate:147, Mate:159, Flush:153, Insert:223, Insert:224, Insert:225, Insert:226, Mate:166, Mate:170, Flush:157, Mate:171, Mate:172, Flush:158, Mate:173, Mate:174, Flush:159, Mate:175, Mate:176, Flush:160, Mate:177, Flush:161, Mate:178, Mate:179, Mate:180, Mate:181, Mate:182, Tangent:89, Tangent:90, Tangent:91, Tangent:92, Tangent:93, Mate:183, Mate:208, Mate:210
467. Hopper Left Side:1 — Mate:140, Flush:81, Mate:142, Mate:143, Flush:83, Flush:84, Mate:145, Mate:146, Insert:210, Insert:211, Insert:212, Insert:213, Insert:214, Mate:156, Mate:152, Insert:217, Insert:218, Insert:219, Insert:220, Insert:221, Insert:222, Mate:154, Mate:157, Flush:152, Insert:264, Insert:265, Insert:266, Mate:185, Insert:275, Insert:276
468. Hopper Back Wedge Side:1 — Mate:141, Mate:142, Flush:82, Flush:151, Mate:184, Mate:186, Flush:162, Insert:267, Insert:268, Insert:269, Insert:270, Insert:271, Insert:272, Insert:273, Insert:274
469. Hopper Top:1 — Mate:144, Flush:83, Flush:84, Mate:167, Insert:215, Insert:216, Mate:162, Mate:163, Mate:169, Insert:243, Insert:244, Insert:245, Insert:246, Insert:247, Insert:248, Insert:249, Mate:196, Mate:197, Mate:198, Mate:199, Angle:76, Mate:215, Angle:78
470. Hopper Left Side Leg:1 — Flush:79, Mate:134, Mate:135, Mate:137, Mate:140, Insert:284, Insert:286, Insert:291, Insert:290
471. Hopper Bracing P2:1 — Mate:130, Mate:133, Flush:79, Mate:134, Insert:328, Insert:329
472. Hopper Bracing P3:1 — Mate:132, Flush:78, Mate:137, Mate:203, Insert:330, Insert:331
473. Hopper Bracing P1:1 — Mate:104, Mate:220, Flush:17, Insert:204, Mate:201, Mate:221, Mate:222, Mate:223, Flush:170, Flush:171
## Relationships (665: Insert 379, Mate 202, Flush 59, Tangent 16, Angle 8, RelateRotation 1)
- Mate:11: Bearing Mount 2 v1:2 ↔ Rebuild Shooter Main Base:1
- Mate:12: Bearing Mount 2 v1:2 ↔ Rebuild Shooter Main Base:1
- Mate:8: Bearing Mount 2 v1:1 ↔ Rebuild Shooter Main Base:1
- Mate:9: Bearing Mount 2 v1:1 ↔ Rebuild Shooter Main Base:1
- [Insert]: Bearing:2 ↔ Bearing Mount 2 v1:2
- [Insert]: Bearing:1 ↔ Bearing Mount 2 v1:1
- [Flush] (-25.4 mm): Bearing:1 ↔ Shorter Shaft:1
- [Mate]: Bearing:1 ↔ Shorter Shaft:1
- [Mate]: Bearing:1 ↔ Shorter Shaft:1
- Mate:10: Bearing Mount 2 v1:1 ↔ Rebuild Shooter Main Base:1
- Mate:13: Bearing Mount 2 v1:2 ↔ Rebuild Shooter Main Base:1
- Mate:14: Bearing Mount 2 v1:1 ↔ Rebuild Shooter Main Base:1
- Mate:19: Bearing:2 ↔ Shorter Shaft:1
- Mate:20: Spur Gear2:1 ↔ Gusset 5:1
- Mate:21: Spur Gear2:1 ↔ Gusset 5:1
- Mate:22: Spur Gear2:1 ↔ Gusset 5:1
- Mate:23: Spur Gear2:1 ↔ Gusset 5:2
- Mate:24: Spur Gear2:1 ↔ Gusset 5:2
- Mate:25: Spur Gear2:1 ↔ Gusset 5:2
- Mate:27: Spur Gear2:1 ↔ Gusset 5:4
- Mate:28: Spur Gear2:1 ↔ Gusset 5:3
- Mate:29: Spur Gear2:1 ↔ Gusset 5:3
- Mate:30: Spur Gear2:1 ↔ Gusset 5:3
- Mate:31: Spur Gear2:1 ↔ Gusset 5:4
- Mate:32: Spur Gear2:1 ↔ Gusset 5:4
- Mate:33: Gusset 5:3 ↔ Rebuild Shooter Main Base:1
- Mate:34: Gusset 5:2 ↔ Rebuild Shooter Main Base:1
- Mate:35: Gusset 5:2 ↔ Rebuild Shooter Main Base:1
- Mate:36: Rebuild L-Channel Strength:1 ↔ Rebuild Shooter Main Base:1
- Mate:37: Rebuild L-Channel Strength:1 ↔ Rebuild Shooter Main Base:1
- Mate:38: Rebuild L-Channel Strength:1 ↔ Rebuild Shooter Main Base:1
- Mate:39: Bearing Mount v1:1 ↔ Rebuild Shooter Main Base:1
- Mate:40: Shooter Back Support Bar:1 ↔ Bearing Mount v1:1
- Flush:2: Bearing Mount v1:1 ↔ Rebuild Shooter Main Base:1
- Mate:41: Bearing Mount v1:1 ↔ Rebuild Shooter Main Base:1
- Mate:42: Rebuild Outer Rail v1:1 ↔ Rebuild Shooter Main Base:1
- Mate:44: Rebuild Outer Rail v1:1 ↔ Bearing Mount v1:1
- Mate:45: Bearing Mount Top:1 ↔ Rebuild Outer Rail v1:1
- Mate:46: Bearing Mount Top:1 ↔ Rebuild Outer Rail v1:1
- Mate:47: Bearing Mount Top:1 ↔ 90630A110:3
- Mate:48: Rubber Cushion:1 ↔ Rebuild Outer Rail v1:1
- Mate:49: Rubber Cushion:1 ↔ Bearing Mount v1:1
- Flush:3 (6.35 mm): Rubber Cushion:1 ↔ Bearing Mount v1:1
- Insert:7: Bearing Mount Top:1 ↔ CIM Bearing:1
- Insert:8: Bearing Mount v1:1 ↔ CIM Bearing:2
- Mate:50: Bearing Mount Top:1 ↔ Pneumatic Wheel:1
- Mate:51: 8mm shaft 2:1 ↔ CIM Bearing:1
- Mate:52: 8mm shaft 2:1 ↔ 2469K200:1
- Mate:53: 2469K200:1 ↔ CIM motor1:1
- Mate:54: 8mm shaft 2:1 ↔ CIM motor1:1
- Flush:4 (-17.2974 mm): 2469K200:1 ↔ CIM motor1:1
- Rotation:1 [RelateRotation] (1 ul): 8mm shaft 2:1 ↔ 2469K200:1
- Insert:9 (8.89 mm): Cim Mount:1 ↔ CIM motor1:1
- Mate:55: Cim Mount:1 ↔ Rebuild Shooter Main Base:1
- Mate:56: Cim Mount:1 ↔ Rebuild Shooter Main Base:1
- Mate:57: Shooter Middle Support Bar:1 ↔ Cim Mount:1
- Mate:58: Cim Mount:1 ↔ CIM motor1:1
- Mate:59: Runner Rails v2:1 ↔ Bearing Mount v1:1
- Mate:60: Runner Rails v2:1 ↔ Bearing Mount v1:1
- Mate:61: Runner Rails v2:1 ↔ Bearing Mount v1:1
- Mate:66: 8mm shaft 2:1 ↔ Pneumatic Hub:1
- Mate:67: 8mm shaft 2:1 ↔ Pneumatic Hub:2
- Mate:68: 8mm shaft 2:1 ↔ Pneumatic Hub:2
- Mate:69: 8mm shaft 2:1 ↔ Pneumatic Hub:1
- Mate:70: Pneumatic Wheel:1 ↔ Pneumatic Hub:2
- Mate:71: Pneumatic Wheel:1 ↔ Pneumatic Hub:1
- Mate:72: Pneumatic Wheel:1 ↔ Pneumatic Hub:2
- Insert:10: 0.25x20 Washer:6 ↔ 0.25x20 Washer:7
- Insert:11: 0.25x20 Washer:7 ↔ 0.25x20 Washer:8
- Insert:12: 0.25x20 Washer:5 ↔ 0.25x20 Washer:8
- Insert:13: 0.25x20 Washer:4 ↔ 0.25x20 Washer:5
- Insert:14: 0.25x20 Washer:1 ↔ 0.25x20 Washer:3
- Insert:15: 0.25x20 Washer:1 ↔ 0.25x20 Washer:2
- Insert:16: 0.25x20 Washer:2 ↔ 0.25x20 Washer:10
- Insert:17: 0.25x20 Washer:9 ↔ 0.25x20 Washer:10
- Insert:18: 0.25x20 Washer:9 ↔ 0.25x20 Washer:12
- Insert:19: 0.25x20 Washer:4 ↔ 0.25x20 Washer:11
- Insert:20: 0.25x20 Washer:12 ↔ 0.25x20 Washer:14
- Insert:21: 0.25x20 Washer:11 ↔ 0.25x20 Washer:13
- Insert:22: Cim Mount:1 ↔ 0.25x20 Washer:14
- Insert:23: Cim Mount:1 ↔ 0.25x20 Washer:13
- Insert:26: 0.25x20 Washer:18 ↔ 0.25x20 Washer:19
- Insert:27: 0.25x20 Washer:19 ↔ 0.25x20 Washer:20
- Insert:28: 0.25x20 Washer:20 ↔ 0.25x20 Washer:21
- Insert:29: 0.25x20 Washer:21 ↔ 0.25x20 Washer:22
- Insert:30: 0.25x20 Washer:17 ↔ 0.25x20 Washer:23
- Insert:31: 0.25x20 Washer:23 ↔ 0.25x20 Washer:24
- Insert:32: 0.25x20 Washer:24 ↔ 0.25x20 Washer:25
- Insert:33: 0.25x20 Washer:25 ↔ 0.25x20 Washer:26
- Insert:34: Cim Mount:1 ↔ 0.25x20 Washer:26
- Insert:35: Cim Mount:1 ↔ 0.25x20 Washer:22
- Insert:39: Rebuild Shooter Main Base:1 ↔ 0.25x20 Washer:31
- Insert:40: Cim Mount:1 ↔ 0.25x20 Washer:27
- Insert:44: Rebuild Shooter Main Base:1 ↔ 0.25x20 Washer:36
- Insert:45: Shooter Middle Support Bar:1 ↔ 0.25x20 Washer:32
- Insert:46: 0.25x20 Washer:91 ↔ 92620A542:1
- Insert:47: 0.25x20 Washer:90 ↔ 92620A542:2
- Insert:48: 0.25x20 Washer:89 ↔ 90630A110:2
- Insert:49: 0.25x20 Washer:88 ↔ 90630A110:1
- Insert:50: 0.25x20 Washer:38 ↔ 0.25x20 Washer:37
- Insert:51: Rebuild Outer Rail v1:1 ↔ 0.25x20 Washer:37
- [Insert]: 0.25x20 Washer:40 ↔ 0.25x20 Washer:39
- Insert:53: Rebuild Outer Rail v1:1 ↔ 0.25x20 Washer:39
- [Insert]: 0.25x20 Washer:42 ↔ 0.25x20 Washer:41
- Insert:55: Rebuild Outer Rail v1:1 ↔ 0.25x20 Washer:41
- Insert:56: Bearing Mount Top:1 ↔ 0.25x20 Washer:43
- Insert:57: Shooter Top Shield:1 ↔ 0.25x20 Washer:44
- Insert:58: Shooter Top Shield:1 ↔ 0.25x20 Washer:45
- Insert:59: 90630A110:4 ↔ 0.25x20 Washer:45
- Insert:60: 90630A110:3 ↔ 0.25x20 Washer:42
- Insert:61: 90630A110:6 ↔ 0.25x20 Washer:40
- Insert:62: 90630A110:5 ↔ 0.25x20 Washer:44
- Insert:63: 90630A110:8 ↔ 0.25x20 Washer:38
- Insert:64: 90630A110:7 ↔ 0.25x20 Washer:43
- Insert:65 (46.8313 mm): Rebuild Shooter Main Base:1 ↔ 92620A559:1
- Insert:66: Bearing Mount v1:1 ↔ 0.25x20 Washer:47
- [Insert]: 92620A557:1 ↔ 0.25x20 Washer:47
- Mate:73: 0.25x20 Washer:46 ↔ 0.25x20 Washer:37
- Mate:74: Rebuild Shooter Main Base:1 ↔ 0.25x20 Washer:46
- [Insert]: 92620A557:2 ↔ 0.25x20 Washer:46
- Insert:69: Rebuild Outer Rail v1:1 ↔ 0.25x20 Washer:48
- Insert:70: 90630A110:9 ↔ 0.25x20 Washer:48
- Insert:71: Cim Mount:1 ↔ 0.25x20 Washer:50
- Insert:72: Cim Mount:1 ↔ 0.25x20 Washer:49
- Insert:73: 90630A110:10 ↔ 0.25x20 Washer:50
- Insert:74: 90630A110:11 ↔ 0.25x20 Washer:49
- Insert:75: 93330A493:1 ↔ Cim Mount:1
- Mate:75: 0.5 inch Shaft to 8mm Shaft Insert:1 ↔ 8mm shaft 2:1
- Mate:76: 0.5 inch Shaft to 8mm Shaft Insert:1 ↔ 8mm shaft 2:1
- Mate:77: 6280K341:1 ↔ 0.5 inch Shaft to 8mm Shaft Insert:1
- Flush:5: 6280K341:1 ↔ 0.5 inch Shaft to 8mm Shaft Insert:1
- Angle:3 (0 deg): 6280K341:1 ↔ 0.5 inch Shaft to 8mm Shaft Insert:1
- Mate:78: 6280K341:1 ↔ 8mm Shaft Spacer 1 Shooter:1
- Mate:79: 8mm Shaft Spacer 1 Shooter:1 ↔ 8mm shaft 2:1
- Mate:80: 8mm Shaft Spacer 1 Shooter:1 ↔ CIM Bearing:1
- Mate:81: Shooter 8mm Key Sprocket Encoder:1 ↔ 8mm shaft 2:1
- Mate:82: Shooter 8mm Key Sprocket Encoder:1 ↔ 8mm shaft 2:1
- Mate:83: 8mm Shaft Spacer 1 Shooter:1 ↔ Shooter 8mm Key Sprocket Encoder:1
- Insert:76: Rebuild Shooter Main Base:1 ↔ 0.25x20 Washer:51
- Insert:77: 92620A555:1 ↔ 0.25x20 Washer:51
- Mate:84: Shooter Side Support Bar - R:1 ↔ Rebuild Shooter Main Base:1
- Tangent:86: Shooter Side Support Bar - R:1 ↔ 0.25x20 Washer:23
- Flush:6: Shooter Side Support Bar - R:1 ↔ Rebuild Shooter Main Base:1
- Mate:85: Shooter Side Support Bar - L:1 ↔ Rebuild Shooter Main Base:1
- Flush:7: Shooter Side Support Bar - L:1 ↔ Rebuild Shooter Main Base:1
- Tangent:87: Shooter Side Support Bar - L:1 ↔ 0.25x20 Washer:31
- Mate:86: Shooter Side Support Bar - R:1 ↔ Shooter Back Support Bar:1
- Tangent:88: Shooter Back Support Bar:1 ↔ 0.25x20 Washer:46
- Flush:8: Shooter Side Support Bar - R:1 ↔ Shooter Back Support Bar:1
- Insert:78: Shooter Side Support Bar - R:1 ↔ 0.25x20 Washer:52
- Insert:79: 0.25x20 Washer:52 ↔ 0.25x20 Washer:53
- Insert:80: 0.25x20 Washer:53 ↔ 0.25x20 Washer:54
- Insert:81: 0.25x20 Washer:54 ↔ 0.25x20 Washer:55
- Insert:82: 0.25x20 Washer:55 ↔ 0.25x20 Washer:56
- Mate:88: Wheel Shield 1:1 ↔ Rebuild L-Channel Strength:1
- Flush:9: Wheel Shield 1:1 ↔ Rebuild L-Channel Strength:1
- Mate:89: Shooter Wheel Shields Connector Bar:1 ↔ Wheel Shield 2:1
- Flush:10: Wheel Shield 2:1 ↔ Wheel Shield 1:1
- Mate:90: Wheel Shield 2:1 ↔ Wheel Shield 1:1
- Flush:11: Wheel Shield 2:1 ↔ Wheel Shield 1:1
- Insert:84: Runner Rails v2:1 ↔ 0.25x20 Washer:57
- Flush:14: Shooter Middle Support Bar:1 ↔ Runner Rails v2:1
- Mate:93: Shooter Middle Support Bar:1 ↔ Cim Mount:1
- Insert:85: Shooter Middle Support Bar:1 ↔ 0.25x20 Washer:58
- Insert:86: Runner Rails v2:1 ↔ 0.25x20 Washer:59
- Insert:87: Shooter Middle Support Bar:1 ↔ 0.25x20 Washer:60
- Insert:88: Runner Rails v2:1 ↔ 0.25x20 Washer:61
- Insert:89: DBK_0820Spacer_am-2243 (modified):1 ↔ 0.25x20 Washer:58
- Insert:90: DBK_0820Spacer_am-2243 (modified):2 ↔ 0.25x20 Washer:60
- Mate:92: DBK_0820Spacer_am-2243 (modified):1 ↔ 0.25x20 Washer:59
- Insert:91: DBK_0820Spacer_am-2243 (modified 2):1 ↔ 0.25x20 Washer:32
- Insert:92: Shooter Side Support Bar - L:1 ↔ 0.25x20 Washer:62
- Insert:93: Cim Mount:1 ↔ Standard #10 Washer:1
- Insert:94: Bearing Mount v1:1 ↔ Standard #10 Washer:2
- Insert:95: Standard #10 Washer:1 ↔ 91735A829:1
- Insert:96: Standard #10 Washer:2 ↔ 91735A829:2
- Insert:100: Shooter Side Support Bar - L:1 ↔ 0.25x20 Washer:63
- Insert:101: Runner Rails v2:1 ↔ 0.25x20 Washer:64
- Insert:102: Runner Rails v2:1 ↔ 0.25x20 Washer:65
- Insert:103: Shooter Middle Support Bar:1 ↔ 0.25x20 Washer:66
- Insert:104: Shooter Middle Support Bar:1 ↔ 0.25x20 Washer:67
- Insert:105: 90630A110:13 ↔ 0.25x20 Washer:66
- Insert:106: 90630A110:14 ↔ 0.25x20 Washer:67
- Insert:107: 92620A546:1 ↔ 0.25x20 Washer:64
- Insert:108: 92620A546:2 ↔ 0.25x20 Washer:65
- Insert:109: 92620A544:1 ↔ 0.25x20 Washer:57
- Insert:110: 0.25x20 Washer:68 ↔ 0.25x20 Washer:17
- Insert:111: 0.25x20 Washer:69 ↔ 0.25x20 Washer:18
- Insert:112: Rebuild Shooter Main Base:1 ↔ 0.25x20 Washer:70
- Insert:113: 90630A110:15 ↔ 0.25x20 Washer:70
- Insert:114: Shooter Side Support Bar - R:1 ↔ 0.25x20 Washer:71
- Insert:115: Shooter Side Support Bar - R:1 ↔ 0.25x20 Washer:72
- Insert:116: Cim Mount:1 ↔ 0.25x20 Washer:73
- Insert:117: Cim Mount:1 ↔ 0.25x20 Washer:74
- Insert:118: 90630A110:16 ↔ 0.25x20 Washer:73
- Insert:119: 90630A110:17 ↔ 0.25x20 Washer:74
- Insert:121: Rebuild L-Channel Strength:1 ↔ 90630A110:19
- Insert:122: Rebuild Shooter Main Base:1 ↔ 92620A548:1
- Insert:123: 0.25x20 Washer Large Diameter:1 ↔ 90630A110:20
- Insert:124: 0.25x20 Washer Large Diameter:1 ↔ 90630A110:21
- Insert:125 (25.4 mm): Rebuild L-Channel Strength:1 ↔ 0.25x20 Washer Large Diameter:1
- Mate:98: 7547K130:1 ↔ Shorter Shaft:1
- Mate:99: 7547K130:1 ↔ Shorter Shaft:1
- Mate:100: 7547K130:1 ↔ Bearing:1
- Mate:101: 7547K130:3 ↔ Shorter Shaft:1
- Mate:102: 7547K130:3 ↔ Shorter Shaft:1
- Mate:103: 7547K130:3 ↔ Bearing:2
- Mate:104: Runner Rails v2:1 ↔ Hopper Bracing P1:1
- Mate:220 (-12.7 mm): Runner Rails v2:1 ↔ Hopper Bracing P1:1
- Flush:17: Runner Rails v2:1 ↔ Hopper Bracing P1:1
- Mate:105: Shooter I Brace:1 ↔ Rebuild Shooter Main Base:1
- Flush:18: Shooter I Brace:1 ↔ Rebuild Shooter Main Base:1
- Insert:127: 0.25x20 Washer:100 ↔ 90630A110:23
- Insert:128: 0.25x20 Washer:101 ↔ 90630A110:24
- Insert:129: 0.25x20 Washer:102 ↔ 90630A110:25
- Insert:130: Shooter Back Support Bar:1 ↔ 0.25x20 Washer:75
- Insert:131: 90630A110:26 ↔ 0.25x20 Washer:76
- Insert:132: 92620A540:1 ↔ 0.25x20 Washer:75
- Insert:133: Bearing Mount 2 v1:2 ↔ 0.25x20 Washer:76
- [Insert]: 92620A540:2 ↔ 0.25x20 Washer:77
- Insert:135: Shooter Side Support Bar - R:1 ↔ 0.25x20 Washer:77
- [Insert]: 90630A110:27 ↔ 0.25x20 Washer:78
- Insert:137: Bearing Mount 2 v1:2 ↔ 0.25x20 Washer:78
- [Insert]: 90630A110:28 ↔ 0.25x20 Washer:79
- Insert:139: Bearing Mount 2 v1:1 ↔ 0.25x20 Washer:79
- [Insert]: 90630A110:29 ↔ 0.25x20 Washer:80
- Insert:141: Gusset 5:3 ↔ 0.25x20 Washer:80
- [Insert]: 90630A110:30 ↔ 0.25x20 Washer:81
- [Insert]: 90630A110:31 ↔ 0.25x20 Washer:82
- [Insert]: 90630A110:32 ↔ 0.25x20 Washer:83
- Insert:145: Gusset 5:2 ↔ 0.25x20 Washer:81
- Insert:146: Gusset 5:4 ↔ 0.25x20 Washer:82
- Insert:147: Gusset 5:1 ↔ 0.25x20 Washer:83
- Insert:148: Rebuild Shooter Main Base:1 ↔ 0.25x20 Washer:84
- Insert:149: Rebuild Shooter Main Base:1 ↔ 0.25x20 Washer:85
- Mate:106: Rebuild Shooter Main Base:1 ↔ 0.25x20 Washer:87
- Mate:107: Rebuild Shooter Main Base:1 ↔ 0.25x20 Washer:86
- Insert:150: Gusset 5:2 ↔ 0.25x20 Washer:89
- Insert:151: Gusset 5:1 ↔ 0.25x20 Washer:88
- Insert:152: Gusset 5:3 ↔ 0.25x20 Washer:90
- Insert:153: Gusset 5:4 ↔ 0.25x20 Washer:91
- Insert:154: 92620A540:3 ↔ 0.25x20 Washer:87
- Insert:155: 92620A540:4 ↔ 0.25x20 Washer:86
- Insert:156: 92620A540:5 ↔ 0.25x20 Washer:85
- Insert:157: 92620A540:6 ↔ 0.25x20 Washer:84
- [Insert]: 92620A540:7 ↔ 0.25x20 Washer:92
- Mate:108: Rebuild Shooter Main Base:1 ↔ 0.25x20 Washer:92
- Mate:109: Shooter I Brace:1 ↔ 0.25x20 Washer:92
- [Insert]: 92620A540:8 ↔ 0.25x20 Washer:93
- Mate:110: Rebuild Shooter Main Base:1 ↔ 0.25x20 Washer:93
- Mate:111: Shooter I Brace:1 ↔ 0.25x20 Washer:93
- [Insert]: 92620A540:9 ↔ 0.25x20 Washer:94
- Mate:112: Rebuild Shooter Main Base:1 ↔ 0.25x20 Washer:94
- Mate:113: Shooter I Brace:1 ↔ 0.25x20 Washer:94
- Insert:161: 91257A544:1 ↔ 0.25x20 Washer:71
- Insert:162: 91257A544:2 ↔ 0.25x20 Washer:72
- Mate:114: Rebuild Outer Rail v1:1 ↔ Rebuild Outer Rail v1:2
- Flush:65: Rebuild Outer Rail v1:1 ↔ Rebuild Outer Rail v1:2
- Flush:66: Rebuild Outer Rail v1:1 ↔ Rebuild Outer Rail v1:2
- Mate:115: Rebuild Outer Rail v1:2 ↔ Rebuild Outer Rail v1:3
- Mate:116: Rebuild Outer Rail v1:3 ↔ Rebuild Outer Rail v1:4
- Mate:117: Rebuild Outer Rail v1:4 ↔ Rebuild Outer Rail v1:5
- Flush:67: Rebuild Outer Rail v1:2 ↔ Rebuild Outer Rail v1:3
- Flush:68: Rebuild Outer Rail v1:3 ↔ Rebuild Outer Rail v1:4
- Flush:69: Rebuild Outer Rail v1:4 ↔ Rebuild Outer Rail v1:5
- Flush:70: Rebuild Outer Rail v1:2 ↔ Rebuild Outer Rail v1:3
- Flush:71: Rebuild Outer Rail v1:3 ↔ Rebuild Outer Rail v1:4
- Flush:72: Rebuild Outer Rail v1:4 ↔ Rebuild Outer Rail v1:5
- Mate:118: Rebuild Outer Rail v1:5 ↔ Bearing Mount v1:1
- Insert:163: Cim Mount:1 ↔ 90630A110:33
- Insert:164: Shooter Middle Support Bar:1 ↔ 92620A537:1
- Insert:165: Bearing Mount v1:1 ↔ 91831A411:1
- Insert:166: Bearing Mount v1:1 ↔ 91831A411:2
- Insert:167: Bearing Mount v1:1 ↔ 91831A411:3